# Autodesk Inventor assembly: ServoAssembly
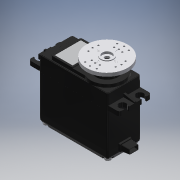
[picture p0: Inventor's stored thumbnail of the model, 180x180]
Saved by Autodesk Inventor 2018 (Build 220112000, 112)
## iProperties
Created: 2019-02-22
Part Number: ServoAssembly
Document SubType Name: Assembly
Designer: snipe
Author: snipe
## Documents named in this file (3)
- C:\Users\snipe\Documents\CPRE186-CAD\ServoAssembly.iam
- C:\Users\snipe\Documents\CPRE186-CAD\Servo.iam
- C:\Users\snipe\Documents\CPRE186-CAD\servoHornRound.ipt
## Components (2 placed, 2 different names)
1. Servo:1 [sub-assembly] — Mate:1, Mate:2
2. servoHornRound:1 — Mate:1, Mate:2
## Relationships (2: Mate 2)
- Mate:1: Servo:1 ↔ servoHornRound:1
- Mate:2: Servo:1 ↔ servoHornRound:1
